# Autodesk Inventor assembly: Front B Battery Pack
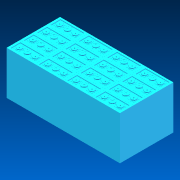
[picture p0: Inventor's stored thumbnail of the model, 180x180]
Saved by Autodesk Inventor 2012 (Build 160160000, 160)
## iProperties
Created: 2012-07-06
Part Number: Front B Battery Pack
Document SubType Name: Assembly
Designer: Hemant
Author: Hemant
## Documents named in this file (2)
- C:\Users\Hemant\Documents\Battery Boxes\Batteries\Front B Battery Pack.iam
- C:\Users\Hemant\Documents\Battery Boxes\Batteries\CALB100AH final.ipt
## Components (16 placed, 1 different names)
1. CALB100AH final:1
2. CALB100AH final:2
3. CALB100AH final:3
4. CALB100AH final:4
5. CALB100AH final:5
6. CALB100AH final:6
7. CALB100AH final:7
8. CALB100AH final:8
9. CALB100AH final:9
10. CALB100AH final:10
11. CALB100AH final:11
12. CALB100AH final:12
13. CALB100AH final:13
14. CALB100AH final:14
15. CALB100AH final:15
16. CALB100AH final:16
## Component patterns: (4 elements), (4 elements, first: CALB100AH final:1), Component Pattern 3:2 (4 elements), Component Pattern 3:3 (4 elements), Component Pattern 3:4 (4 elements)
